# Autodesk Inventor assembly: Head
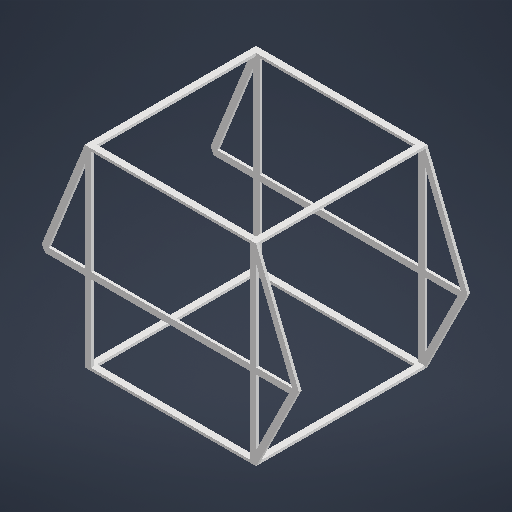
[picture p0: Inventor's stored thumbnail of the model, 512x512]
Saved by Autodesk Inventor 2026 (Build 300175000, 175)
## iProperties
Created: 2025-09-02
Part Number: Head
Document SubType Name: Assembly
Designer: trott
Author: trott
## Documents named in this file (7)
- C:\Users\trott\Documents\UofSC-ASME-Tiger-Burn-Design-2025\CAD\Head\Head.iam
- C:\Users\trott\Documents\UofSC-ASME-Tiger-Burn-Design-2025\CAD\Head\2x4x96.ipt
- C:\Users\trott\Documents\UofSC-ASME-Tiger-Burn-Design-2025\CAD\Head\2x4x89.ipt
- C:\Users\trott\Documents\UofSC-ASME-Tiger-Burn-Design-2025\CAD\Head\2x4x105.ipt
- C:\Users\trott\Documents\UofSC-ASME-Tiger-Burn-Design-2025\CAD\Head\S_2x4x24.ipt
- C:\Users\trott\Documents\UofSC-ASME-Tiger-Burn-Design-2025\CAD\Head\S_2x4x64.622.ipt
- C:\Users\trott\Documents\UofSC-ASME-Tiger-Burn-Design-2025\CAD\Head\S_2x4x48.13.ipt
## Components (24 placed, 6 different names)
1. 2x4x89:5 — Mate:5, Flush:11, Flush:12, Flush:14, Flush:15, Flush:18, Flush:23, Flush:24
2. 2x4x89:6 — Mate:6, Flush:13, Flush:14
3. S_2x4x64.622:1 — Mate:9, Flush:19
4. S_2x4x64.622:2 — Mate:10, Flush:20
5. S_2x4x64.622:3 — Mate:11, Mate:12, Flush:21
6. S_2x4x64.622:4 — Mate:13, Mate:14
7. S_2x4x48.13:1 — Mate:15, Flush:22, Mate:16
8. S_2x4x48.13:2 — Mate:17, Flush:25
9. 2x4x105:1 — Mate:4, Flush:9, Flush:10, Mate:5, Flush:11, Mate:8, Flush:17
10. 2x4x105:2 — Mate:6, Flush:13
11. 2x4x105:3 — Mate:7, Flush:16, Flush:22
12. 2x4x105:4 — Flush:25
13. 2x4x96:1 — Mate:1, Flush:1, Flush:2, Mate:2, Flush:3, Flush:4, Mate:4, Flush:9, Flush:10
14. 2x4x89:1 — Mate:1, Flush:1, Flush:2, Flush:8
15. 2x4x89:2 — Mate:2, Flush:3, Flush:4, Flush:5, Mate:3, Flush:6, Flush:7, Flush:12
16. 2x4x96:2 — Flush:5, Mate:3, Flush:6, Flush:7, Flush:8, Mate:15, Mate:16
17. 2x4x96:3 — Mate:12, Mate:13
18. 2x4x89:3
19. 2x4x89:4
20. 2x4x96:4
21. S_2x4x24:2 — Mate:8, Flush:17, Flush:18, Mate:11, Flush:21, Flush:24
22. S_2x4x24:1 — Mate:7, Flush:15, Flush:16, Mate:10, Flush:20, Flush:23
23. S_2x4x24:3 — Mate:14
24. S_2x4x24:4 — Mate:9, Flush:19, Mate:17
## Component patterns: (4 elements, first: 2x4x105:1), (2 elements, first: 2x4x96:1 + 2x4x89:1 + 2x4x89:2 + 2x4x96:2), (2 elements, first: S_2x4x24:2 + S_2x4x24:1)
## Relationships (42: Flush 25, Mate 17)
- Mate:1: 2x4x96:1 ↔ 2x4x89:1
- Flush:1: 2x4x96:1 ↔ 2x4x89:1
- Flush:2: 2x4x96:1 ↔ 2x4x89:1
- Mate:2: 2x4x96:1 ↔ 2x4x89:2
- Flush:3: 2x4x96:1 ↔ 2x4x89:2
- Flush:4: 2x4x96:1 ↔ 2x4x89:2
- Flush:5: 2x4x89:2 ↔ 2x4x96:2
- Mate:3: 2x4x89:2 ↔ 2x4x96:2
- Flush:6: 2x4x89:2 ↔ 2x4x96:2
- Flush:7: 2x4x89:2 ↔ 2x4x96:2
- Flush:8: 2x4x89:1 ↔ 2x4x96:2
- Mate:4: 2x4x105:1 ↔ 2x4x96:1
- Flush:9: 2x4x105:1 ↔ 2x4x96:1
- Flush:10: 2x4x105:1 ↔ 2x4x96:1
- Mate:5: 2x4x89:5 ↔ 2x4x105:1
- Flush:11: 2x4x89:5 ↔ 2x4x105:1
- Flush:12 (1130.3 mm): 2x4x89:5 ↔ 2x4x89:2
- Mate:6: 2x4x89:6 ↔ 2x4x105:2
- Flush:13: 2x4x89:6 ↔ 2x4x105:2
- Flush:14: 2x4x89:5 ↔ 2x4x89:6
- Mate:7: 2x4x105:3 ↔ S_2x4x24:1
- Flush:15: 2x4x89:5 ↔ S_2x4x24:1
- Flush:16: 2x4x105:3 ↔ S_2x4x24:1
- Mate:8: 2x4x105:1 ↔ S_2x4x24:2
- Flush:17: 2x4x105:1 ↔ S_2x4x24:2
- Flush:18: 2x4x89:5 ↔ S_2x4x24:2
- Mate:9: S_2x4x64.622:1 ↔ S_2x4x24:4
- Flush:19: S_2x4x64.622:1 ↔ S_2x4x24:4
- Mate:10: S_2x4x64.622:2 ↔ S_2x4x24:1
- Flush:20: S_2x4x64.622:2 ↔ S_2x4x24:1
- Mate:11: S_2x4x64.622:3 ↔ S_2x4x24:2
- Mate:12: S_2x4x64.622:3 ↔ 2x4x96:3
- Flush:21: S_2x4x64.622:3 ↔ S_2x4x24:2
- Mate:13: S_2x4x64.622:4 ↔ 2x4x96:3
- Mate:14: S_2x4x64.622:4 ↔ S_2x4x24:3
- Mate:15: S_2x4x48.13:1 ↔ 2x4x96:2
- Flush:22: S_2x4x48.13:1 ↔ 2x4x105:3
- Mate:16: S_2x4x48.13:1 ↔ 2x4x96:2
- Flush:23: 2x4x89:5 ↔ S_2x4x24:1
- Flush:24: 2x4x89:5 ↔ S_2x4x24:2
- Mate:17: S_2x4x48.13:2 ↔ S_2x4x24:4
- Flush:25: S_2x4x48.13:2 ↔ 2x4x105:4
